# Autodesk Inventor assembly: Two Eyes
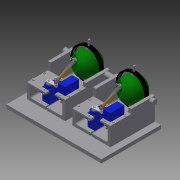
[picture p0: Inventor's stored thumbnail of the model, 180x180]
Saved by Autodesk Inventor 2013 (Build 170138000, 138)
## iProperties
Created: 2012-10-31
Part Number: Two Eyes
Document SubType Name: Assembly
Designer: uqgtayle
Author: uqgtayle
## Documents named in this file (3)
- G:\workshops-design\Mechanical\2012 Jobs\Grant\Animatronic Eyes\Two Eyes.iam
- G:\workshops-design\Mechanical\2012 Jobs\Grant\Animatronic Eyes\Base Plate.ipt
- G:\workshops-design\Mechanical\2012 Jobs\Grant\Animatronic Eyes\Eyes.iam
## Components (3 placed, 2 different names)
1. Base Plate:1 — Mate:1, Mate:2, Flush:1, Flush:2, Flush:3, Flush:4
2. Eyes:1 [sub-assembly] — Mate:1, Flush:1, Flush:3
3. Eyes:2 [sub-assembly] — Mate:2, Flush:2, Flush:4
## Relationships (6: Flush 4, Mate 2)
- Mate:1: Base Plate:1 ↔ Eyes:1
- Mate:2: Base Plate:1 ↔ Eyes:2
- Flush:1: Base Plate:1 ↔ Eyes:1
- Flush:2: Base Plate:1 ↔ Eyes:2
- Flush:3 (10 mm): Base Plate:1 ↔ Eyes:1
- Flush:4 (-10 mm): Base Plate:1 ↔ Eyes:2
